# Autodesk Inventor assembly: turret_assembly
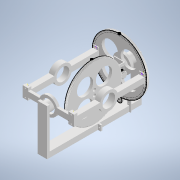
[picture p0: Inventor's stored thumbnail of the model, 180x180]
Saved by Autodesk Inventor 2021 (Build 250183000, 183)
## iProperties
Created: 2020-09-03
Part Number: turret_assembly
Document SubType Name: Assembly
Designer: bober
Author: bober
## Documents named in this file (8)
- D:\Turret\Models\turret_assembly.iam
- D:\Turret\Models\turret_assembly\Design Accelerator\vertical_axis_small_gear.ipt
- D:\Turret\Models\turret_assembly\Design Accelerator\vertical_axis_bigl_gear.ipt
- D:\Turret\Models\turret_assembly\Design Accelerator\horizontal_axis_big_gear.ipt
- D:\Turret\Models\turret_assembly\Design Accelerator\pylon.ipt
- D:\Turret\Models\turret_assembly\Design Accelerator\upper_grip.ipt
- D:\Turret\Models\turret_assembly\Design Accelerator\main_stand_lower_half.ipt
- D:\Turret\Models\turret_assembly\Design Accelerator\main_stand_upper_half.ipt
## Components (9 placed, 7 different names)
1. vertical_axis_small_gear:1 — Rotational:3
2. horizontal_axis_big_gear:1
3. vertical_axis_small_gear:2 — Rotational:2
4. vertical_axis_bigl_gear:2 — Rigid:2, Rigid:3, Rotational:2
5. pylon:1 — Rigid:2
6. pylon:2 — Rigid:3, Rotational:1
7. upper_grip:1 — Rotational:1
8. main_stand_lower_half:1 — Rotational:3, Rotational:4
9. main_stand_upper_half:1 — Rotational:4
## Relationships (6: RevoluteJoint 4, WeldJoint 2)
- Rigid:2 [WeldJoint]: vertical_axis_bigl_gear:2 ↔ pylon:1
- Rigid:3 [WeldJoint]: vertical_axis_bigl_gear:2 ↔ pylon:2
- Rotational:1 [RevoluteJoint]: pylon:2 ↔ upper_grip:1
- Rotational:2 [RevoluteJoint]: vertical_axis_small_gear:2 ↔ vertical_axis_bigl_gear:2
- Rotational:3 [RevoluteJoint]: vertical_axis_small_gear:1 ↔ main_stand_lower_half:1
- Rotational:4 [RevoluteJoint]: main_stand_lower_half:1 ↔ main_stand_upper_half:1
